# Autodesk Inventor assembly: Lifting Assy
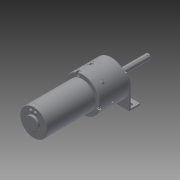
[picture p0: Inventor's stored thumbnail of the model, 180x180]
Saved by Autodesk Inventor 2015 (Build 190159000, 159)
## iProperties
Created: 2015-02-10
Part Number: Lifting Assy
Document SubType Name: Assembly
Designer: pltwe4
Author: pltwe4
## Documents named in this file (3)
- C:\Users\pltwe4\Documents\recycling-rush\model\Lifting Assy.iam
- C:\Users\pltwe4\Documents\recycling-rush\model\3_stageGEM.iam
- C:\Users\pltwe4\Documents\recycling-rush\model\CIM Bracket.ipt
## Components (2 placed, 2 different names)
1. 3_stageGEM:1 [sub-assembly] — Mate:4, Mate:5
2. CIM Bracket:1 — Mate:1, Mate:2, Mate:3, Mate:4, Mate:5
## Relationships (5: Mate 5)
- Mate:1: CIM Bracket:1
- Mate:2: CIM Bracket:1
- Mate:3: CIM Bracket:1
- Mate:4: 3_stageGEM:1 ↔ CIM Bracket:1
- Mate:5: 3_stageGEM:1 ↔ CIM Bracket:1
